# Autodesk Inventor assembly: engranajes motor hombro dimer 3.1
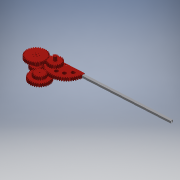
[picture p0: Inventor's stored thumbnail of the model, 180x180]
Saved by Autodesk Inventor 2016 (Build 200138000, 138)
## iProperties
Created: 2016-06-23
Part Number: engranajes motor hombro dimer 3.1
Document SubType Name: Assembly
Designer: Admin
Author: Admin
## Documents named in this file (12)
- C:\Users\Admin\Dropbox\diseños autodesk dimer\engranajes dimer hombro muelles\engranajes motor hombro dimer 3.1.iam
- C:\Users\Admin\Dropbox\piezas 3d dimer\engranajes motor hombro dimer 3.1\Design Accelerator\Spur Gears1.iam
- C:\Users\Admin\Dropbox\piezas 3d dimer\engranajes motor hombro dimer 3.1\Design Accelerator\Spur Gears3.iam
- C:\Users\Admin\Dropbox\diseños autodesk dimer\engranajes dimer hombro muelles\perfil aluminio.ipt
- C:\Users\Admin\Dropbox\diseños autodesk dimer\engranajes dimer hombro muelles\caja perfil.ipt
- C:\Users\Admin\Dropbox\diseños autodesk dimer\engranajes dimer hombro muelles\eje motor.ipt
- C:\Users\Admin\Dropbox\diseños autodesk dimer\engranajes dimer hombro muelles\engranajes motor hombro dimer 3.1\Design Accelerator\Spur Gears1.iam
- C:\Users\Admin\Dropbox\diseños autodesk dimer\engranajes dimer hombro muelles\engranajes motor hombro dimer 3.1\Design Accelerator\Spur Gears2.iam
- C:\Users\Admin\Dropbox\diseños autodesk dimer\engranajes dimer hombro muelles\eje union engrane reductor.ipt
- C:\Users\Admin\Dropbox\diseños autodesk dimer\engranajes dimer hombro muelles\engranajes motor hombro dimer 3.1\Design Accelerator\Spur Gear11.ipt
- C:\Users\Admin\Dropbox\piezas 3d dimer\engranajes motor hombro dimer 3.1\Design Accelerator\Spur Gear23.ipt
- C:\Users\Admin\Dropbox\diseños autodesk dimer\engranajes dimer hombro muelles\engranaje gusano.ipt
## Components (13 placed, 12 different names)
1. piñon motor [sub-assembly] — Flush:7, Mate:4, Tangent:1, Rotation:1, Mate:9
2. engrane brazo [sub-assembly] — Mate:2, Flush:3, Flush:9
3. perfil aluminio:1 — Flush:4, Flush:5, Flush:6, Mate:12
4. caja perfil:1 — Mate:2, Flush:3, Flush:4, Flush:5, Flush:6
5. eje motor:1 — Flush:7, Mate:4
6. reductor motor [sub-assembly] — Mate:5, Mate:6, Mate:7, Tangent:1, Rotation:1, Mate:9
7. reductor brazo [sub-assembly] — Mate:5, Mate:6, Mate:8, Flush:8
8. eje union engrane reductor:1 — Mate:7, Mate:8
9. reductor 31 — Mate:10, Mate:11, Flush:8
10. reductor32 [sub-assembly] — Mate:10, Mate:11, Flush:9
11. Spur Gear2:1 — Mate:12, Flush:14, Mate:14, Flush:15
12. caja perfil:2 — Flush:14, Mate:14, Flush:15
13. engranaje gusano:1
## Relationships (22: Mate 11, Flush 9, Tangent 1, RelateRotation 1)
- Mate:2 (-8.5 mm): engrane brazo ↔ caja perfil:1
- Flush:3: engrane brazo ↔ caja perfil:1
- Flush:4 (2.5 mm): perfil aluminio:1 ↔ caja perfil:1
- Flush:5 (2.5 mm): perfil aluminio:1 ↔ caja perfil:1
- Flush:6 (-417 mm): perfil aluminio:1 ↔ caja perfil:1
- Flush:7: piñon motor ↔ eje motor:1
- Mate:4: piñon motor ↔ eje motor:1
- Mate:5: reductor motor ↔ reductor brazo
- Mate:6 (26 mm): reductor motor ↔ reductor brazo
- Mate:7: reductor motor ↔ eje union engrane reductor:1
- Tangent:1: piñon motor ↔ reductor motor
- Rotation:1 [RelateRotation] (1 ul): piñon motor ↔ reductor motor
- Mate:8: reductor brazo ↔ eje union engrane reductor:1
- Mate:9 (-15 mm): piñon motor ↔ reductor motor
- Mate:10: reductor 31 ↔ reductor32
- Mate:11: reductor 31 ↔ reductor32
- Flush:8: reductor brazo ↔ reductor 31
- Flush:9: engrane brazo ↔ reductor32
- Mate:12 (250 mm): perfil aluminio:1 ↔ Spur Gear2:1
- Flush:14: Spur Gear2:1 ↔ caja perfil:2
- Mate:14: Spur Gear2:1 ↔ caja perfil:2
- Flush:15 (-6 mm): Spur Gear2:1 ↔ caja perfil:2
